# Autodesk Inventor assembly: Existing_Basement_And_Transition
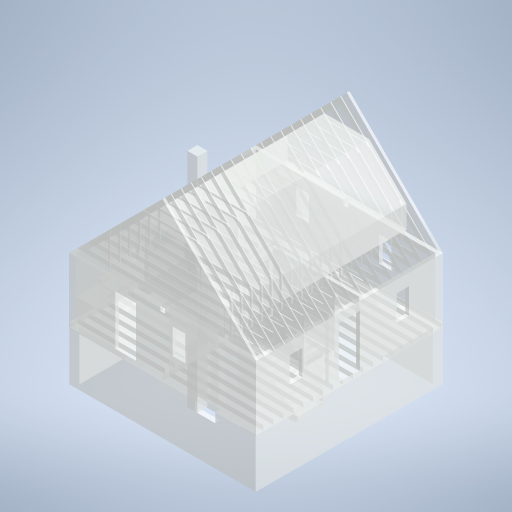
[picture p0: Inventor's stored thumbnail of the model, 512x512]
Saved by Autodesk Inventor 2024 (Build 280153000, 153)
## iProperties
Created: 2023-05-19
Part Number: Existing_Basement_And_Transition
Document SubType Name: Assembly
Designer: Tom
Author: Tom
## Documents named in this file (6)
- C:\Users\Tom\Documents\Tom_Levers_Public_Git_Repository\Inventor\Mobility\Existing_House.iam
- C:\Users\Tom\Documents\Tom_Levers_Public_Git_Repository\Inventor\Mobility\Basement\Existing_Basement.iam
- C:\Users\Tom\Documents\Tom_Levers_Public_Git_Repository\Inventor\Mobility\Transition_For_Existing_Basement_And_First_Floor.ipt
- C:\Users\Tom\Documents\Tom_Levers_Public_Git_Repository\Inventor\Mobility\First_Floor\Existing_First_Floor.iam
- C:\Users\Tom\Documents\Tom_Levers_Public_Git_Repository\Inventor\Mobility\Attic\Existing_Attic.iam
- C:\Users\Tom\Documents\Tom_Levers_Public_Git_Repository\Inventor\Mobility\First_Floor\Stairs_Between_First_Floor_And_Second_Floor.ipt
## Components (5 placed, 5 different names)
1. Existing_Basement:1 [sub-assembly] — Mate:1, Flush:1, Flush:2, Flush:3
2. Transition_For_Existing_Basement_And_First_Floor:1 — Mate:1, Flush:1, Flush:2, Mate:2, Flush:4, Mate:7
3. Existing_First_Floor:1 [sub-assembly] — Mate:2, Flush:3, Flush:4, Flush:5, Mate:3, Mate:5, Mate:6
4. Existing_Attic:1 [sub-assembly] — Flush:5, Mate:3, Mate:4
5. Stairs_Between_First_Floor_And_Second_Floor:1 — Mate:5, Mate:6, Mate:7
## Relationships (12: Mate 7, Flush 5)
- Mate:1: Existing_Basement:1 ↔ Transition_For_Existing_Basement_And_First_Floor:1
- Flush:1: Existing_Basement:1 ↔ Transition_For_Existing_Basement_And_First_Floor:1
- Flush:2 (-215.9 mm): Existing_Basement:1 ↔ Transition_For_Existing_Basement_And_First_Floor:1
- Mate:2: Transition_For_Existing_Basement_And_First_Floor:1 ↔ Existing_First_Floor:1
- Flush:3: Existing_Basement:1 ↔ Existing_First_Floor:1
- Flush:4: Transition_For_Existing_Basement_And_First_Floor:1 ↔ Existing_First_Floor:1
- Flush:5: Existing_First_Floor:1 ↔ Existing_Attic:1
- Mate:3: Existing_First_Floor:1 ↔ Existing_Attic:1
- Mate:4: Existing_Attic:1
- Mate:5: Existing_First_Floor:1 ↔ Stairs_Between_First_Floor_And_Second_Floor:1
- Mate:6: Existing_First_Floor:1 ↔ Stairs_Between_First_Floor_And_Second_Floor:1
- Mate:7: Transition_For_Existing_Basement_And_First_Floor:1 ↔ Stairs_Between_First_Floor_And_Second_Floor:1
## Named parameters: sa_0 = 980.999, sa_1 = 19.1674, sa_2 = 19.1674
note: some values were not read from the file. Shown as the stored number, unit unknown: "sa_0", "sa_1", "sa_2".
